# Autodesk Inventor assembly: Beam Splitter
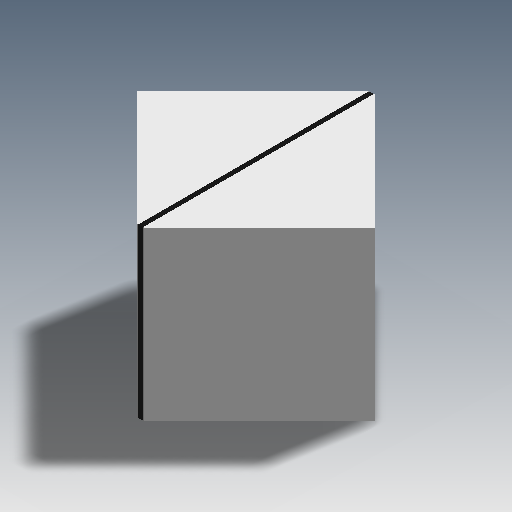
[picture p0: Inventor's stored thumbnail of the model, 512x512]
Saved by Autodesk Inventor 2026 (Build 300175050, 175E)
## iProperties
Created: 2025-08-02
Part Number: Beam Splitter
Document SubType Name: Assembly
Designer: aman0
Author: aman0
## Documents named in this file (3)
- D:\Academics\Projects\Physics Enabled Raytracer\Code\Models\Inventor Files\Beam Splitter.iam
- D:\Academics\Projects\Physics Enabled Raytracer\Code\Models\Inventor Files\Beamsplittertransparent.ipt
- D:\Academics\Projects\Physics Enabled Raytracer\Code\Models\Inventor Files\BeamsplitterReflect.ipt
## Components (2 placed, 2 different names)
1. Beamsplittertransparent:1 — Angle:1, Angle:2, Mate:1, Flush:1, Flush:2
2. BeamsplitterReflect:1 — Mate:1, Flush:1, Flush:2
## Relationships (5: Angle 2, Flush 2, Mate 1)
- Angle:1 (0 deg): Beamsplittertransparent:1
- Angle:2 (45 deg): Beamsplittertransparent:1
- Mate:1: Beamsplittertransparent:1 ↔ BeamsplitterReflect:1
- Flush:1: Beamsplittertransparent:1 ↔ BeamsplitterReflect:1
- Flush:2: Beamsplittertransparent:1 ↔ BeamsplitterReflect:1
